# Autodesk Inventor assembly: Randverbinder lang
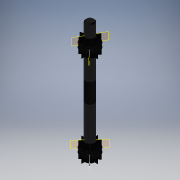
[picture p0: Inventor's stored thumbnail of the model, 180x180]
Saved by Autodesk Inventor 2019 (Build 230136000, 136)
## iProperties
Created: 2019-11-23
Part Number: Randverbinder lang
Material: Generisch
Document SubType Name: Assembly
Designer: seele
Author: seele
## Documents named in this file (3)
- I:\Desktop\Neuer Ordner\Randverbinder lang.iam
- I:\Desktop\Neuer Ordner\Randverbinder lang.ipt
- I:\Desktop\Neuer Ordner\Randverbinder2.ipt
## Components (5 placed, 2 different names)
1. Randverbinder lang:1 — Passend:1, Passend:2, Passend:3, Passend:4, Fluchtend:1, Passend:7
2. Randverbinder2:1 — Passend:1, Passend:6, Passend:7
3. Randverbinder2:2 — Passend:2, Passend:6
4. Randverbinder2:3 — Passend:4, Fluchtend:1, Passend:5
5. Randverbinder2:4 — Passend:3, Passend:5
## Relationships (8: Mate 7, Flush 1)
- Passend:1 [Mate]: Randverbinder lang:1 ↔ Randverbinder2:1
- Passend:2 [Mate]: Randverbinder lang:1 ↔ Randverbinder2:2
- Passend:3 [Mate]: Randverbinder lang:1 ↔ Randverbinder2:4
- Passend:4 [Mate]: Randverbinder lang:1 ↔ Randverbinder2:3
- Fluchtend:1 [Flush]: Randverbinder lang:1 ↔ Randverbinder2:3
- Passend:5 [Mate] (16 mm): Randverbinder2:3 ↔ Randverbinder2:4
- Passend:6 [Mate] (16 mm): Randverbinder2:1 ↔ Randverbinder2:2
- Passend:7 [Mate] (-88 mm): Randverbinder lang:1 ↔ Randverbinder2:1
